# Autodesk Inventor assembly: pcb
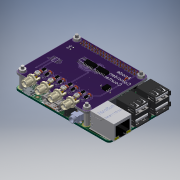
[picture p0: Inventor's stored thumbnail of the model, 180x180]
Saved by Autodesk Inventor 2016 (Build 200138000, 138)
## iProperties
Created: 2016-06-27
Part Number: pcb
Document SubType Name: Assembly
Designer: Jonathan
Author: Jonathan
## Documents named in this file (18)
- C:\Users\Jonathan\Documents\Projects\anodePiShield\coincidenceCounter\cad\pcb.iam
- C:\Users\Jonathan\Documents\Projects\anodePiShield\coincidenceCounter\cad\Board.ipt
- C:\Users\Jonathan\Documents\Projects\anodePiShield\coincidenceCounter\cad\electronics\PVZ3A\PVZ3A.iam
- C:\Users\Jonathan\Documents\Projects\anodePiShield\coincidenceCounter\cad\electronics\SOT23-6.ipt
- C:\Users\Jonathan\Documents\Projects\anodePiShield\coincidenceCounter\cad\electronics\soic\soic-8-N.ipt
- C:\Users\Jonathan\Documents\Projects\anodePiShield\coincidenceCounter\cad\electronics\soic\soic.ipt
- C:\Users\Jonathan\Documents\Projects\anodePiShield\coincidenceCounter\cad\electronics\soic\soic-14-N.ipt
- C:\Users\Jonathan\Documents\Projects\anodePiShield\coincidenceCounter\cad\electronics\SMA Female Edge Mount CONSMA003-062.ipt
- C:\Users\Jonathan\Documents\Projects\anodePiShield\coincidenceCounter\cad\electronics\resistor\chipResistor\chipResistor-0402.ipt
- C:\Users\Jonathan\Documents\Projects\anodePiShield\coincidenceCounter\cad\wire.ipt
- C:\Users\Jonathan\Documents\Projects\anodePiShield\coincidenceCounter\cad\electronics\capacitor\capacitor-0402.ipt
- C:\Users\Jonathan\Documents\Projects\anodePiShield\coincidenceCounter\cad\electronics\capacitor\capacitor.ipt
- C:\Users\Jonathan\Documents\Projects\anodePiShield\coincidenceCounter\cad\electronics\resistor\chipResistor.ipt
- C:\Users\Jonathan\Documents\Projects\anodePiShield\coincidenceCounter\cad\electronics\femaleHeaders\femaleHeaders.iam
- C:\Users\Jonathan\Documents\Projects\anodePiShield\coincidenceCounter\cad\electronics\raspberrypi_b_+_(assembly).ipt
- C:\Users\Jonathan\Documents\Projects\anodePiShield\coincidenceCounter\cad\hardware\11mm M2.5 standoff.ipt
- C:\Users\Jonathan\Documents\Projects\anodePiShield\coincidenceCounter\cad\hardware\M2.5 hex nut.ipt
- C:\Users\Jonathan\Documents\Projects\anodePiShield\coincidenceCounter\cad\hardware\M2.5 6mm screw.ipt
## Components (57 placed, 14 different names)
1. Board:1 — Angle:2, Mate:2, Mate:3, Mate:4, Angle:3, Angle:4, Mate:5, Mate:6, Mate:7, Mate:8, Mate:9, Mate:10, Mate:11, Mate:12, Mate:13, Mate:14, Mate:16, Mate:17, Mate:18, Mate:19, Mate:20, Mate:21, Mate:22, Mate:23, Mate:28, Mate:29, Mate:30, Mate:31
2. PVZ3A:1 [sub-assembly] — Flush:3, Flush:6
3. PVZ3A:2 [sub-assembly] — Flush:2, Flush:3, Flush:5, Flush:6
4. PVZ3A:3 [sub-assembly] — Flush:1, Flush:2, Flush:4, Flush:5
5. PVZ3A:4 [sub-assembly] — Angle:2, Flush:1, Flush:4, Mate:2
6. SOT23-6:1 — Flush:9, Flush:15
7. SOT23-6:2 — Flush:8, Flush:9, Flush:14, Flush:15
8. SOT23-6:3 — Flush:7, Flush:8, Flush:13, Flush:14
9. SOT23-6:4 — Flush:7, Flush:13, Flush:19
10. SOT23-6:5 — Flush:12, Flush:18
11. SOT23-6:6 — Flush:11, Flush:12, Flush:17, Flush:18
12. SOT23-6:7 — Flush:10, Flush:11, Flush:16, Flush:17
13. SOT23-6:8 — Flush:10, Flush:16, Flush:19, Mate:3
14. soic-8-N:1 — Mate:4
15. soic-14-N:2 — Angle:4, Flush:20, Flush:21
16. soic-14-N:3 — Angle:3, Flush:20, Flush:21, Mate:5
17. SMA Female Edge Mount CONSMA003-062:1 — Flush:22, Flush:23, Flush:25, Flush:26
18. SMA Female Edge Mount CONSMA003-062:2 — Flush:23, Flush:24, Flush:26, Flush:27
19. SMA Female Edge Mount CONSMA003-062:3 — Flush:24, Flush:27
20. SMA Female Edge Mount CONSMA003-062:4 — Flush:22, Flush:25, Mate:6, Mate:7
21. chipResistor-0402:1
22. chipResistor-0402:2
23. chipResistor-0402:3 — Mate:11
24. chipResistor-0402:4
25. chipResistor-0402:5
26. chipResistor-0402:6
27. chipResistor-0402:7
28. chipResistor-0402:8 — Mate:10
29. chipResistor-0402:9
30. chipResistor-0402:10
31. chipResistor-0402:11
32. chipResistor-0402:12 — Mate:9
33. wire:1 — Mate:8
34. wire:2 — Flush:53, Flush:54
35. wire:3 — Flush:59, Mate:12
36. wire:4 — Flush:53
37. wire:5 — Flush:55, Flush:56
38. wire:6 — Flush:54, Flush:55
39. wire:7 — Flush:56, Flush:57
40. wire:8 — Flush:58, Flush:59
41. wire:9 — Flush:57, Flush:58
42. capacitor-0402:1 — Flush:60
43. capacitor-0402:2 — Flush:60, Mate:13
44. femaleHeaders:1 [sub-assembly] — Mate:14, Mate:15
45. raspberrypi_b_+_(assembly):1 — Mate:15, Angle:12, Mate:32, Mate:33, Mate:38, Mate:39, Mate:40, Mate:41
46. 11mm M2.5 standoff:1 — Mate:16, Mate:20, Mate:25, Angle:8, Angle:10, Mate:37, Angle:13
47. 11mm M2.5 standoff:2 — Mate:17, Mate:22, Mate:26, Angle:11, Mate:33, Mate:34, Angle:15
48. 11mm M2.5 standoff:3 — Mate:18, Mate:21, Mate:27, Angle:9, Mate:32, Mate:35, Angle:14
49. 11mm M2.5 standoff:4 — Mate:19, Mate:23, Mate:24, Angle:10, Angle:11, Angle:12, Mate:36, Angle:16
50. M2.5 hex nut:1 — Mate:25, Mate:29, Angle:7, Angle:8, Angle:9
51. M2.5 hex nut:2 — Mate:24, Mate:30, Angle:5, Angle:6
52. M2.5 hex nut:3 — Mate:26, Mate:31, Angle:5
53. M2.5 hex nut:4 — Mate:27, Mate:28, Angle:6, Angle:7
54. M2.5 6mm screw:1 — Mate:34, Mate:39, Angle:15
55. M2.5 6mm screw:2 — Mate:36, Mate:40, Angle:16
56. M2.5 6mm screw:3 — Mate:37, Mate:41, Angle:13
57. M2.5 6mm screw:4 — Mate:35, Mate:38, Angle:14
## Relationships (115: Flush 60, Mate 40, Angle 15)
- Angle:2 (0 deg): Board:1 ↔ PVZ3A:4
- Flush:1: PVZ3A:3 ↔ PVZ3A:4
- Flush:2: PVZ3A:2 ↔ PVZ3A:3
- Flush:3: PVZ3A:1 ↔ PVZ3A:2
- Flush:4: PVZ3A:3 ↔ PVZ3A:4
- Flush:5: PVZ3A:2 ↔ PVZ3A:3
- Flush:6: PVZ3A:1 ↔ PVZ3A:2
- Mate:2: Board:1 ↔ PVZ3A:4
- Flush:7: SOT23-6:3 ↔ SOT23-6:4
- Flush:8: SOT23-6:2 ↔ SOT23-6:3
- Flush:9: SOT23-6:1 ↔ SOT23-6:2
- Flush:10: SOT23-6:7 ↔ SOT23-6:8
- Flush:11: SOT23-6:6 ↔ SOT23-6:7
- Flush:12: SOT23-6:5 ↔ SOT23-6:6
- Flush:13: SOT23-6:3 ↔ SOT23-6:4
- Flush:14: SOT23-6:2 ↔ SOT23-6:3
- Flush:15: SOT23-6:1 ↔ SOT23-6:2
- Flush:16: SOT23-6:7 ↔ SOT23-6:8
- Flush:17: SOT23-6:6 ↔ SOT23-6:7
- Flush:18: SOT23-6:5 ↔ SOT23-6:6
- Flush:19: SOT23-6:4 ↔ SOT23-6:8
- Mate:3: Board:1 ↔ SOT23-6:8
- Mate:4: Board:1 ↔ soic-8-N:1
- Angle:3 (0 deg): Board:1 ↔ soic-14-N:3
- Angle:4 (0 deg): Board:1 ↔ soic-14-N:2
- Flush:20: soic-14-N:2 ↔ soic-14-N:3
- Flush:21: soic-14-N:2 ↔ soic-14-N:3
- Mate:5: Board:1 ↔ soic-14-N:3
- Flush:22: SMA Female Edge Mount CONSMA003-062:1 ↔ SMA Female Edge Mount CONSMA003-062:4
- Flush:23: SMA Female Edge Mount CONSMA003-062:1 ↔ SMA Female Edge Mount CONSMA003-062:2
- Flush:24: SMA Female Edge Mount CONSMA003-062:2 ↔ SMA Female Edge Mount CONSMA003-062:3
- Flush:25: SMA Female Edge Mount CONSMA003-062:1 ↔ SMA Female Edge Mount CONSMA003-062:4
- Flush:26: SMA Female Edge Mount CONSMA003-062:1 ↔ SMA Female Edge Mount CONSMA003-062:2
- Flush:27: SMA Female Edge Mount CONSMA003-062:2 ↔ SMA Female Edge Mount CONSMA003-062:3
- Mate:6: Board:1 ↔ SMA Female Edge Mount CONSMA003-062:4
- Mate:7: Board:1 ↔ SMA Female Edge Mount CONSMA003-062:4
- [Flush]: chipResistor-0402:2 ↔ chipResistor-0402:3
- [Flush]: chipResistor-0402:1 ↔ chipResistor-0402:2
- [Flush]: chipResistor-0402:2 ↔ chipResistor-0402:3
- [Flush]: chipResistor-0402:3 ↔ chipResistor-0402:4
- [Flush]: chipResistor-0402:1 ↔ chipResistor-0402:2
- [Flush]: chipResistor-0402:3 ↔ chipResistor-0402:4
- [Flush]: chipResistor-0402:6 ↔ chipResistor-0402:7
- [Flush]: chipResistor-0402:5 ↔ chipResistor-0402:6
- [Flush]: chipResistor-0402:6 ↔ chipResistor-0402:7
- [Flush]: chipResistor-0402:7 ↔ chipResistor-0402:8
- [Flush]: chipResistor-0402:5 ↔ chipResistor-0402:6
- [Flush]: chipResistor-0402:7 ↔ chipResistor-0402:8
- [Flush]: chipResistor-0402:10 ↔ chipResistor-0402:11
- [Flush]: chipResistor-0402:9 ↔ chipResistor-0402:10
- [Flush]: chipResistor-0402:10 ↔ chipResistor-0402:11
- [Flush]: chipResistor-0402:11 ↔ chipResistor-0402:12
- [Flush]: chipResistor-0402:9 ↔ chipResistor-0402:10
- [Flush]: chipResistor-0402:11 ↔ chipResistor-0402:12
- Mate:8: Board:1 ↔ wire:1
- Mate:9: Board:1 ↔ chipResistor-0402:12
- Mate:10: Board:1 ↔ chipResistor-0402:8
- Mate:11: Board:1 ↔ chipResistor-0402:3
- [Flush]: wire:2 ↔ wire:3
- [Flush]: wire:2 ↔ wire:4
- [Flush]: wire:4 ↔ wire:6
- [Flush]: wire:6 ↔ wire:8
- [Flush]: wire:3 ↔ wire:5
- [Flush]: wire:5 ↔ wire:7
- [Flush]: wire:7 ↔ wire:9
- Flush:53: wire:2 ↔ wire:4
- Flush:54: wire:2 ↔ wire:6
- Flush:55: wire:5 ↔ wire:6
- Flush:56: wire:5 ↔ wire:7
- Flush:57: wire:7 ↔ wire:9
- Flush:58: wire:8 ↔ wire:9
- Flush:59: wire:3 ↔ wire:8
- Mate:12: Board:1 ↔ wire:3
- Flush:60: capacitor-0402:1 ↔ capacitor-0402:2
- Mate:13: Board:1 ↔ capacitor-0402:2
- Mate:14: Board:1 ↔ femaleHeaders:1
- Mate:15: femaleHeaders:1 ↔ raspberrypi_b_+_(assembly):1
- Mate:16: Board:1 ↔ 11mm M2.5 standoff:1
- Mate:17: Board:1 ↔ 11mm M2.5 standoff:2
- Mate:18: Board:1 ↔ 11mm M2.5 standoff:3
- Mate:19: Board:1 ↔ 11mm M2.5 standoff:4
- Mate:20: Board:1 ↔ 11mm M2.5 standoff:1
- Mate:21: Board:1 ↔ 11mm M2.5 standoff:3
- Mate:22: Board:1 ↔ 11mm M2.5 standoff:2
- Mate:23: Board:1 ↔ 11mm M2.5 standoff:4
- Mate:24: 11mm M2.5 standoff:4 ↔ M2.5 hex nut:2
- Mate:25: 11mm M2.5 standoff:1 ↔ M2.5 hex nut:1
- Mate:26: 11mm M2.5 standoff:2 ↔ M2.5 hex nut:3
- Mate:27: 11mm M2.5 standoff:3 ↔ M2.5 hex nut:4
- Mate:28: Board:1 ↔ M2.5 hex nut:4
- Mate:29: Board:1 ↔ M2.5 hex nut:1
- Mate:30: Board:1 ↔ M2.5 hex nut:2
- Mate:31: Board:1 ↔ M2.5 hex nut:3
- Angle:5 (0 deg): M2.5 hex nut:2 ↔ M2.5 hex nut:3
- Angle:6 (0 deg): M2.5 hex nut:2 ↔ M2.5 hex nut:4
- Angle:7 (0 deg): M2.5 hex nut:1 ↔ M2.5 hex nut:4
- Angle:8 (0 deg): 11mm M2.5 standoff:1 ↔ M2.5 hex nut:1
- Angle:9 (0 deg): 11mm M2.5 standoff:3 ↔ M2.5 hex nut:1
- Angle:10 (0 deg): 11mm M2.5 standoff:1 ↔ 11mm M2.5 standoff:4
- Angle:11 (0 deg): 11mm M2.5 standoff:2 ↔ 11mm M2.5 standoff:4
- Angle:12 (0 deg): raspberrypi_b_+_(assembly):1 ↔ 11mm M2.5 standoff:4
- Mate:32: raspberrypi_b_+_(assembly):1 ↔ 11mm M2.5 standoff:3
- Mate:33: raspberrypi_b_+_(assembly):1 ↔ 11mm M2.5 standoff:2
- Mate:34: 11mm M2.5 standoff:2 ↔ M2.5 6mm screw:1
- Mate:35: 11mm M2.5 standoff:3 ↔ M2.5 6mm screw:4
- Mate:36: 11mm M2.5 standoff:4 ↔ M2.5 6mm screw:2
- Mate:37: 11mm M2.5 standoff:1 ↔ M2.5 6mm screw:3
- Mate:38: raspberrypi_b_+_(assembly):1 ↔ M2.5 6mm screw:4
- Mate:39: raspberrypi_b_+_(assembly):1 ↔ M2.5 6mm screw:1
- Mate:40: raspberrypi_b_+_(assembly):1 ↔ M2.5 6mm screw:2
- Mate:41: raspberrypi_b_+_(assembly):1 ↔ M2.5 6mm screw:3
- Angle:13 (0 deg): 11mm M2.5 standoff:1 ↔ M2.5 6mm screw:3
- Angle:14 (0 deg): 11mm M2.5 standoff:3 ↔ M2.5 6mm screw:4
- Angle:15 (0 deg): 11mm M2.5 standoff:2 ↔ M2.5 6mm screw:1
- Angle:16 (0 deg): 11mm M2.5 standoff:4 ↔ M2.5 6mm screw:2
## Named parameters: d93_d90 = 0 mm, d94_d91 = 0 mm, d95_d40 = 0 mm, d96_d53 = 0 mm, d97_d54 = 0 mm, d98_d55 = 0 mm, d99_d90 = 0 mm, d100_d91 = 0 mm, d101_d40 = 0 mm, d102_d53 = 0 mm, d103_d54 = 0 mm, d104_d55 = 0 mm, d74_d40 = 0 mm
